# Autodesk Inventor assembly: 射出_上部
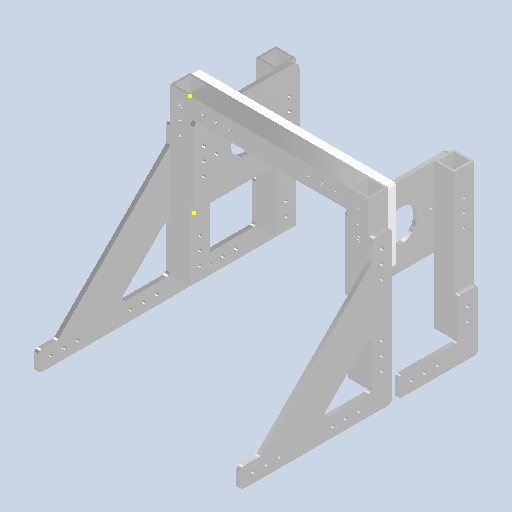
[picture p0: Inventor's stored thumbnail of the model, 512x512]
Saved by Autodesk Inventor 2023 (Build 270158000, 158)
## iProperties
Created: 2022-04-24
Part Number: 射出_上部
Document SubType Name: Assembly
Designer: yuta
Author: yuta
## Documents named in this file (4)
- C:\Users\yuta\Documents\NHK\射出_上部.iam
- C:\Users\yuta\Documents\NHK\射出_受け身.iam
- C:\Users\yuta\Documents\NHK\射出_ベアリング3.iam
- C:\Users\yuta\Documents\NHK\射出_ベアリング2.iam
## Components (3 placed, 3 different names)
1. 射出_受け身:1 [sub-assembly] — メイト:1, フラッシュ:1, フラッシュ:2, メイト:2, メイト:3, フラッシュ:3
2. 射出_ベアリング3:1 [sub-assembly] — メイト:2, メイト:3, フラッシュ:3
3. 射出_ベアリング2:1 [sub-assembly] — メイト:1, フラッシュ:1, フラッシュ:2
## Relationships (6: Mate 3, Flush 3)
- メイト:1 [Mate]: 射出_受け身:1 ↔ 射出_ベアリング2:1
- フラッシュ:1 [Flush]: 射出_受け身:1 ↔ 射出_ベアリング2:1
- フラッシュ:2 [Flush]: 射出_受け身:1 ↔ 射出_ベアリング2:1
- メイト:2 [Mate]: 射出_受け身:1 ↔ 射出_ベアリング3:1
- メイト:3 [Mate]: 射出_受け身:1 ↔ 射出_ベアリング3:1
- フラッシュ:3 [Flush]: 射出_受け身:1 ↔ 射出_ベアリング3:1
